# Autodesk Inventor assembly: Purge Bucket
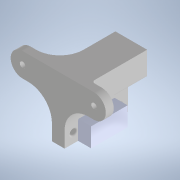
[picture p0: Inventor's stored thumbnail of the model, 180x180]
Saved by Autodesk Inventor 2021 (Build 250183000, 183)
## iProperties
Created: 2021-08-18
Part Number: Purge Bucket
Document SubType Name: Assembly
Designer: Diego.labarca
Author: Diego.labarca
## Documents named in this file (3)
- E:\Dropbox\Inventor\Impresora 3D\Arreglos Impresora\Purge Slide\Purge Bucket.iam
- E:\Dropbox\Inventor\Impresora 3D\Arreglos Impresora\Purge Slide\SG90.ipt
- E:\Dropbox\Inventor\Impresora 3D\Arreglos Impresora\Purge Slide\Soporte MG90S.ipt
## Components (2 placed, 2 different names)
1. SG90:1 — Coincidencia:1, Coincidencia:2, Nivelación:4
2. Soporte MG90S:1 — Nivelación:3, Coincidencia:1, Coincidencia:2, Nivelación:4
## Relationships (4: Flush 2, Mate 2)
- Nivelación:3 [Flush]: Soporte MG90S:1
- Coincidencia:1 [Mate]: SG90:1 ↔ Soporte MG90S:1
- Coincidencia:2 [Mate]: SG90:1 ↔ Soporte MG90S:1
- Nivelación:4 [Flush]: SG90:1 ↔ Soporte MG90S:1
